# Autodesk Inventor assembly: motor_base_cent
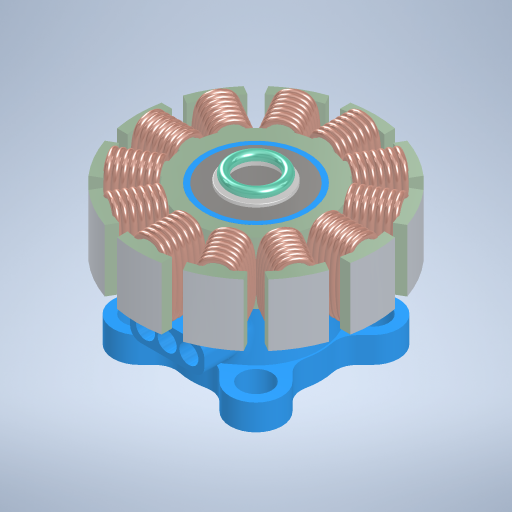
[picture p0: Inventor's stored thumbnail of the model, 512x512]
Saved by Autodesk Inventor 2024 (Build 280153000, 153)
## iProperties
Created: 2024-03-12
Part Number: motor_base_cent
Document SubType Name: Assembly
Designer: nicoe
Mass: 19.4848 g
Surface Area: 62.1049 cm^2
Volume: 2.48214 cm^3
Density: 7.85 g/cm^3
Author: nicoe
## Documents named in this file (2)
- D:\users\nicoe\OneDrive\OneDrive - Stellenbosch University\Desktop\Nico_Masters\1. Drone Constrution\CAD Files\iflight xing-e 2306(To replace R5)\Broken up motor\motor_base_cent.iam
- D:\users\nicoe\OneDrive\OneDrive - Stellenbosch University\Desktop\Nico_Masters\1. Drone Constrution\CAD Files\iflight xing-e 2306(To replace R5)\Broken up motor\motor_base.iam
## Components (1 placed, 1 different names)
1. motor_base:1 [sub-assembly] — Mate:1, Mate:2, Flush:1
## Relationships (3: Mate 2, Flush 1)
- Mate:1: motor_base:1
- Mate:2: motor_base:1
- Flush:1: motor_base:1
